# Autodesk Inventor assembly: Octohedron
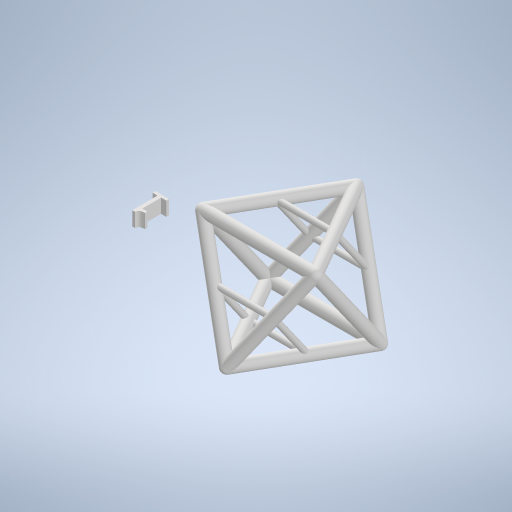
[picture p0: Inventor's stored thumbnail of the model, 512x512]
Saved by Autodesk Inventor 2023 (Build 270158000, 158)
## iProperties
Created: 2023-02-28
Part Number: Octohedron
Document SubType Name: Assembly
Designer: 100KStarsun
Author: 100KStarsun
## Documents named in this file (3)
- C:\Users\100ks\Documents\cwru\Think[Box]\Wire Octohedron\Octohedron.iam
- C:\Users\100ks\Documents\cwru\Think[Box]\Wire Octohedron\Pyramid.iam
- C:\Users\100ks\Documents\cwru\Think[Box]\Wire Octohedron\Text1.ipt
## Components (3 placed, 2 different names)
1. Pyramid:1 [sub-assembly] — Cylindrical:1, Mate:1
2. Pyramid:2 [sub-assembly] — Cylindrical:1, Mate:1
3. Text1:1
## Relationships (2: CylindricalJoint 1, Mate 1)
- Cylindrical:1: Pyramid:1 ↔ Pyramid:2
- Mate:1: Pyramid:1 ↔ Pyramid:2
